# Autodesk Inventor assembly: Full_Stethoscope_Body
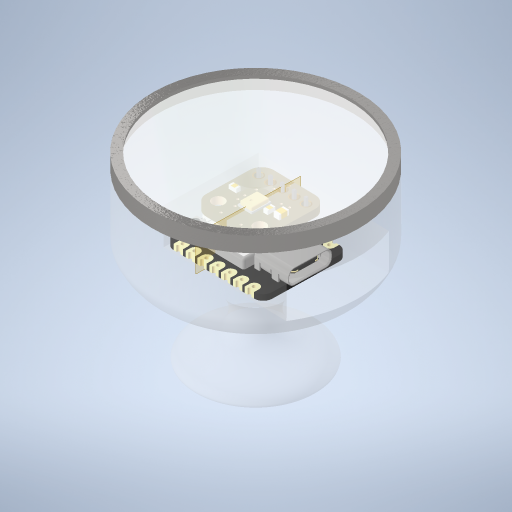
[picture p0: Inventor's stored thumbnail of the model, 512x512]
Saved by Autodesk Inventor 2023.1 (Build 271208000, 208)
## iProperties
Created: 2022-12-07
Part Number: Full_Stethoscope_Body
Document SubType Name: Assembly
Designer: maste
Author: maste
## Documents named in this file (7)
- C:\Users\mnelyubo\Documents\GitHub\Remote-Stethoscope\3D_models\Full_Stethoscope_Body.iam
- C:\Users\mnelyubo\Documents\GitHub\Remote-Stethoscope\3D_models\adafruit_3492\PDM Mic.iam
- C:\Users\mnelyubo\Documents\GitHub\Remote-Stethoscope\3D_models\xiao_rp2040\Seeed Studio XIAO RP2040 v26.iam
- C:\Users\mnelyubo\Documents\GitHub\Remote-Stethoscope\3D_models\IC_pin.ipt
- C:\Users\mnelyubo\Documents\GitHub\Remote-Stethoscope\3D_models\Stacked_Case.ipt
- C:\Users\mnelyubo\Documents\GitHub\Remote-Stethoscope\3D_models\Diaphragm_Ring.ipt
- C:\Users\mnelyubo\Documents\GitHub\Remote-Stethoscope\3D_models\Diaphragm_Film.ipt
## Components (10 placed, 6 different names)
1. PDM Mic:1 [sub-assembly] — Flush:1, Flush:2, Flush:3, Flush:4, Flush:5, Mate:8, Mate:14, Mate:16
2. Seeed Studio XIAO RP2040 v26:1 [sub-assembly] — Mate:7, Mate:8, Mate:9, Mate:10, Mate:11, Mate:12, Mate:13, Mate:17
3. IC_pin:1 — Flush:2, Mate:12, Mate:24, Mate:25
4. IC_pin:2 — Flush:1, Mate:7, Mate:13, Mate:25
5. IC_pin:3 — Flush:3, Mate:11, Mate:14, Mate:15, Mate:23, Mate:24
6. IC_pin:4 — Flush:4, Mate:10, Mate:22, Mate:23
7. IC_pin:5 — Flush:5, Mate:9, Mate:22
8. Stacked_Case:1 — Mate:15, Mate:16, Mate:17, Mate:20, Mate:21
9. Diaphragm_Ring:1 — Mate:18, Mate:19, Mate:20, Mate:21
10. Diaphragm_Film:1 — Mate:18, Mate:19
## Relationships (24: Mate 19, Flush 5)
- Flush:1 (-1.27 mm): PDM Mic:1 ↔ IC_pin:2
- Flush:2 (-1.27 mm): PDM Mic:1 ↔ IC_pin:1
- Flush:3 (-1.27 mm): PDM Mic:1 ↔ IC_pin:3
- Flush:4 (-1.27 mm): PDM Mic:1 ↔ IC_pin:4
- Flush:5 (-1.27 mm): PDM Mic:1 ↔ IC_pin:5
- Mate:7: Seeed Studio XIAO RP2040 v26:1 ↔ IC_pin:2
- Mate:8 (1.27 mm): PDM Mic:1 ↔ Seeed Studio XIAO RP2040 v26:1
- Mate:9: Seeed Studio XIAO RP2040 v26:1 ↔ IC_pin:5
- Mate:10: Seeed Studio XIAO RP2040 v26:1 ↔ IC_pin:4
- Mate:11: Seeed Studio XIAO RP2040 v26:1 ↔ IC_pin:3
- Mate:12: Seeed Studio XIAO RP2040 v26:1 ↔ IC_pin:1
- Mate:13: Seeed Studio XIAO RP2040 v26:1 ↔ IC_pin:2
- Mate:14: PDM Mic:1 ↔ IC_pin:3
- Mate:15: IC_pin:3 ↔ Stacked_Case:1
- Mate:16 (0.254 mm): PDM Mic:1 ↔ Stacked_Case:1
- Mate:17: Seeed Studio XIAO RP2040 v26:1 ↔ Stacked_Case:1
- Mate:18: Diaphragm_Ring:1 ↔ Diaphragm_Film:1
- Mate:19: Diaphragm_Ring:1 ↔ Diaphragm_Film:1
- Mate:20: Stacked_Case:1 ↔ Diaphragm_Ring:1
- Mate:21: Stacked_Case:1 ↔ Diaphragm_Ring:1
- Mate:22: IC_pin:4 ↔ IC_pin:5
- Mate:23: IC_pin:3 ↔ IC_pin:4
- Mate:24: IC_pin:1 ↔ IC_pin:3
- Mate:25: IC_pin:1 ↔ IC_pin:2
